# Autodesk Inventor assembly: Сборка РБАСУ
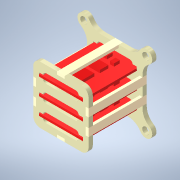
[picture p0: Inventor's stored thumbnail of the model, 180x180]
Saved by Autodesk Inventor 2022 (Build 260153000, 153)
## iProperties
Created: 2022-05-03
Part Number: Сборка РБАСУ
Document SubType Name: Assembly
Designer: Кочетов.А.И.
Author: Кочетов.А.И.
## Documents named in this file (5)
- C:\Users\BornO\Documents\Inventor\БАСУ\РБАСУ\Сборка РБАСУ.iam
- C:\Users\BornO\Documents\Inventor\БАСУ\РБАСУ\Крепление РБАСУ.ipt
- C:\Users\BornO\Documents\Inventor\БАСУ\РБАСУ\РБАСУ.ipt
- C:\Users\BornO\Documents\Inventor\БАСУ\РБАСУ\Балка РБАСУ.ipt
- C:\Users\BornO\Documents\Inventor\БАСУ\РБАСУ\Крепление РБАСУ нижнее.ipt
## Components (11 placed, 4 different names)
1. Крепление РБАСУ:1 — Совмещение:1, Совмещение:2, Совмещение:3, Совмещение:4, Совмещение:5, Совмещение:6, Совмещение:7, Совмещение:8, Совмещение:9, Совмещение:10, Совмещение:11, Совмещение:12, Совмещение:13, Совмещение:14, Совмещение:15, Совмещение:16, Совмещение:17, Совмещение:18, Совмещение:19, Совмещение:20, Совмещение:21, Совмещение:22, Заподлицо:1, Заподлицо:2, Заподлицо:3, Заподлицо:4, Заподлицо:5, Заподлицо:6, Заподлицо:8, Заподлицо:9, Заподлицо:10
2. РБАСУ:1 — Совмещение:4, Совмещение:5, Совмещение:10, Заподлицо:10
3. РБАСУ:2 — Совмещение:8, Совмещение:9, Заподлицо:8
4. РБАСУ:3 — Совмещение:6, Совмещение:7, Заподлицо:9
5. Балка РБАСУ:1 — Совмещение:17, Совмещение:18, Заподлицо:6
6. Балка РБАСУ:2 — Совмещение:19, Совмещение:21, Заподлицо:2
7. Балка РБАСУ:3 — Совмещение:12, Совмещение:15, Заподлицо:4
8. Балка РБАСУ:4 — Совмещение:13, Совмещение:14, Заподлицо:5
9. Балка РБАСУ:5 — Совмещение:11, Совмещение:16, Заподлицо:1, Совмещение:23, Совмещение:24, Заподлицо:11
10. Балка РБАСУ:6 — Совмещение:20, Совмещение:22, Заподлицо:3
11. Крепление РБАСУ нижнее:1 — Совмещение:23, Совмещение:24, Заподлицо:11
## Relationships (34: Mate 24, Flush 10)
- Совмещение:1 [Mate]: Крепление РБАСУ:1
- Совмещение:2 [Mate]: Крепление РБАСУ:1
- Совмещение:3 [Mate]: Крепление РБАСУ:1
- Совмещение:4 [Mate]: Крепление РБАСУ:1 ↔ РБАСУ:1
- Совмещение:5 [Mate]: Крепление РБАСУ:1 ↔ РБАСУ:1
- Совмещение:6 [Mate]: Крепление РБАСУ:1 ↔ РБАСУ:3
- Совмещение:7 [Mate]: Крепление РБАСУ:1 ↔ РБАСУ:3
- Совмещение:8 [Mate]: Крепление РБАСУ:1 ↔ РБАСУ:2
- Совмещение:9 [Mate]: Крепление РБАСУ:1 ↔ РБАСУ:2
- Совмещение:10 [Mate]: Крепление РБАСУ:1 ↔ РБАСУ:1
- Совмещение:11 [Mate]: Крепление РБАСУ:1 ↔ Балка РБАСУ:5
- Совмещение:12 [Mate]: Крепление РБАСУ:1 ↔ Балка РБАСУ:3
- Совмещение:13 [Mate]: Крепление РБАСУ:1 ↔ Балка РБАСУ:4
- Совмещение:14 [Mate]: Крепление РБАСУ:1 ↔ Балка РБАСУ:4
- Совмещение:15 [Mate]: Крепление РБАСУ:1 ↔ Балка РБАСУ:3
- Совмещение:16 [Mate]: Крепление РБАСУ:1 ↔ Балка РБАСУ:5
- Совмещение:17 [Mate]: Крепление РБАСУ:1 ↔ Балка РБАСУ:1
- Совмещение:18 [Mate]: Крепление РБАСУ:1 ↔ Балка РБАСУ:1
- Совмещение:19 [Mate]: Крепление РБАСУ:1 ↔ Балка РБАСУ:2
- Совмещение:20 [Mate]: Крепление РБАСУ:1 ↔ Балка РБАСУ:6
- Совмещение:21 [Mate]: Крепление РБАСУ:1 ↔ Балка РБАСУ:2
- Совмещение:22 [Mate]: Крепление РБАСУ:1 ↔ Балка РБАСУ:6
- Заподлицо:1 [Flush]: Крепление РБАСУ:1 ↔ Балка РБАСУ:5
- Заподлицо:2 [Flush]: Крепление РБАСУ:1 ↔ Балка РБАСУ:2
- Заподлицо:3 [Flush]: Крепление РБАСУ:1 ↔ Балка РБАСУ:6
- Заподлицо:4 [Flush]: Крепление РБАСУ:1 ↔ Балка РБАСУ:3
- Заподлицо:5 [Flush]: Крепление РБАСУ:1 ↔ Балка РБАСУ:4
- Заподлицо:6 [Flush]: Крепление РБАСУ:1 ↔ Балка РБАСУ:1
- Заподлицо:8 [Flush]: Крепление РБАСУ:1 ↔ РБАСУ:2
- Заподлицо:9 [Flush]: Крепление РБАСУ:1 ↔ РБАСУ:3
- Заподлицо:10 [Flush]: Крепление РБАСУ:1 ↔ РБАСУ:1
- Совмещение:23 [Mate]: Балка РБАСУ:5 ↔ Крепление РБАСУ нижнее:1
- Совмещение:24 [Mate]: Балка РБАСУ:5 ↔ Крепление РБАСУ нижнее:1
- Заподлицо:11 [Flush]: Балка РБАСУ:5 ↔ Крепление РБАСУ нижнее:1
